# Autodesk Inventor assembly: Wago 74-831 (32A) Block
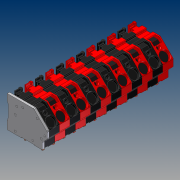
[picture p0: Inventor's stored thumbnail of the model, 180x180]
Saved by Autodesk Inventor 2012 (Build 160160000, 160)
## iProperties
Company: Team 801
Created: 2007-09-01
Part Number: Wago 74-831 (32A) Block
Document SubType Name: Assembly
Designer: Jeffrey M
Catalog Web Link: www.team801.org
Mass: 46.4551 g
Surface Area: 284.607 cm^2
Volume: 46.4551 cm^3
Density: 1 g/cm^3
Author: Jeffrey M
## Documents named in this file (4)
- Z:\UserData\Documents\Inventor\team1885frc\Electronics\PowerDistributionBoard\Wago 745-831 (32A) Block.iam
- Z:\UserData\Documents\Inventor\team1885frc\Electronics\PowerDistributionBoard\Wago 745-831 (32A) Black.ipt
- Z:\UserData\Documents\Inventor\team1885frc\Electronics\PowerDistributionBoard\Wago 745-831 (32A) Red.ipt
- Z:\UserData\Documents\Inventor\team1885frc\Electronics\PowerDistributionBoard\Wago 745-300.ipt
## Components (13 placed, 2 different names)
1. 745-300:1 — Mate:2, Flush:4, Flush:5
2. Wago 745-831 (32A):1 — Mate:1, Flush:1, Flush:2, Mate:2, Flush:4, Flush:5
3. Wago 745-831 (32A):2 — Mate:1, Flush:1, Flush:2
4. Wago 745-831 (32A):3
5. Wago 745-831 (32A):4
6. Wago 745-831 (32A):5
7. Wago 745-831 (32A):6
8. Wago 745-831 (32A):7
9. Wago 745-831 (32A):8
10. Wago 745-831 (32A):9
11. Wago 745-831 (32A):10
12. Wago 745-831 (32A):11
13. Wago 745-831 (32A):12
## Component patterns: (6 elements, first: Wago 745-831 (32A):1 + Wago 745-831 (32A):2)
## Relationships (6: Flush 4, Mate 2)
- Mate:1: Wago 745-831 (32A):1 ↔ Wago 745-831 (32A):2
- Flush:1: Wago 745-831 (32A):1 ↔ Wago 745-831 (32A):2
- Flush:2: Wago 745-831 (32A):1 ↔ Wago 745-831 (32A):2
- Mate:2: 745-300:1 ↔ Wago 745-831 (32A):1
- Flush:4: 745-300:1 ↔ Wago 745-831 (32A):1
- Flush:5: 745-300:1 ↔ Wago 745-831 (32A):1
